# Autodesk Inventor assembly: ASY GBK короткая стенка
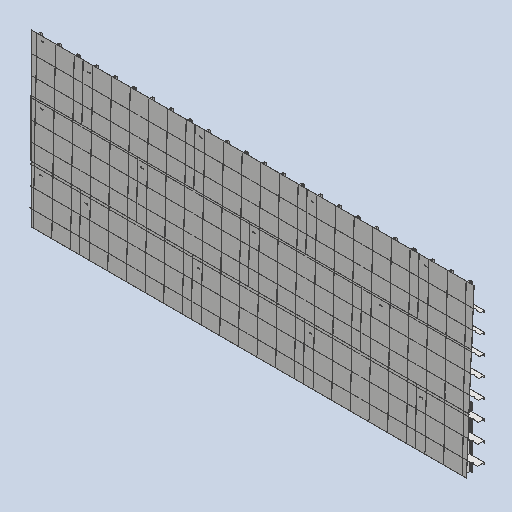
[picture p0: Inventor's stored thumbnail of the model, 512x512]
Saved by Autodesk Inventor 2026.3 (Build 303398000, 398)
## iProperties
Created: 2026-05-24
Part Number: ASY GBK короткая стенка
Document SubType Name: Assembly
Designer: pokla
Mass: 2.92121e+06 g
Surface Area: 1.88753e+06 cm^2
Volume: 372128 cm^3
Density: 7.85 g/cm^3
Stock Number: 2000
Author: pokla
## Documents named in this file (10)
- C:\Users\admin\Documents\Inventor\GBK-Gubkinskiy\ASY GBK короткая стенка.iam
- C:\Users\admin\Documents\Inventor\GBK-Gubkinskiy\ASY GBK 2110 short wall shield 1.iam
- C:\Users\admin\Documents\Inventor\GBK-Gubkinskiy\ASY GBK 2120 short wall shield 2.iam
- C:\Users\admin\Documents\Inventor\GBK-Gubkinskiy\ASY GBK 2130 short wall shield 3.iam
- C:\Users\admin\Documents\Inventor\GBK-Gubkinskiy\ASY GBK 2210 short wall shield 4.iam
- C:\Users\admin\Documents\Inventor\GBK-Gubkinskiy\ASY GBK 2310 short wall shield 7.iam
- C:\Users\admin\Documents\Inventor\GBK-Gubkinskiy\ASY GBK 2320 short wall shield 8.iam
- C:\Users\admin\Documents\Inventor\GBK-Gubkinskiy\ASY GBK 2330 short wall shield 9.iam
- C:\Users\admin\Documents\Inventor\GBK-Gubkinskiy\ASY GBK 2220 short wall shield 5.iam
- C:\Users\admin\Documents\Inventor\GBK-Gubkinskiy\ASY GBK 2230 short wall shield 6.iam
## Components (14 placed, 9 different names)
1. ASY GBK 2110 short wall shield 1:1 [sub-assembly] — Rigid:1, Flush:1, Flush:2, Mate:1
2. ASY GBK 2120 short wall shield 2:1 [sub-assembly] — Rigid:1, Rigid:2
3. ASY GBK 2120 short wall shield 2:2 [sub-assembly] — Rigid:2, Rigid:3
4. ASY GBK 2120 short wall shield 2:3 [sub-assembly] — Rigid:3, Rigid:14
5. ASY GBK 2130 short wall shield 3:1 [sub-assembly] — Rigid:14, Flush:3, Mate:2, Mate:4
6. ASY GBK 2210 short wall shield 4:1 [sub-assembly] — Rigid:17
7. ASY GBK 2220 short wall shield 5:1 [sub-assembly] — Rigid:7, Rigid:17
8. ASY GBK 2220 short wall shield 5:2 [sub-assembly] — Rigid:7, Rigid:16
9. ASY GBK 2230 short wall shield 6:1 [sub-assembly] — Flush:3, Mate:2, Flush:5, Mate:3, Mate:4, Mate:5, Rigid:16
10. ASY GBK 2310 short wall shield 7:1 [sub-assembly] — Rigid:10
11. ASY GBK 2320 short wall shield 8:1 [sub-assembly] — Rigid:10, Rigid:11
12. ASY GBK 2330 short wall shield 9:1 [sub-assembly] — Flush:5, Mate:3, Mate:5, Rigid:15
13. ASY GBK 2320 short wall shield 8:2 [sub-assembly] — Rigid:11, Rigid:12
14. ASY GBK 2320 short wall shield 8:3 [sub-assembly] — Rigid:12, Rigid:15
## Relationships (20: WeldJoint 11, Mate 5, Flush 4)
- Rigid:1 [WeldJoint] (1 mm): ASY GBK 2110 short wall shield 1:1 ↔ ASY GBK 2120 short wall shield 2:1
- Rigid:2 [WeldJoint] (1 mm): ASY GBK 2120 short wall shield 2:1 ↔ ASY GBK 2120 short wall shield 2:2
- Rigid:3 [WeldJoint] (1 mm): ASY GBK 2120 short wall shield 2:2 ↔ ASY GBK 2120 short wall shield 2:3
- Rigid:7 [WeldJoint] (1 mm): ASY GBK 2220 short wall shield 5:1 ↔ ASY GBK 2220 short wall shield 5:2
- Rigid:10 [WeldJoint] (1 mm): ASY GBK 2310 short wall shield 7:1 ↔ ASY GBK 2320 short wall shield 8:1
- Rigid:11 [WeldJoint] (1 mm): ASY GBK 2320 short wall shield 8:1 ↔ ASY GBK 2320 short wall shield 8:2
- Rigid:12 [WeldJoint] (1 mm): ASY GBK 2320 short wall shield 8:2 ↔ ASY GBK 2320 short wall shield 8:3
- Flush:1: ASY GBK 2110 short wall shield 1:1
- Flush:2: ASY GBK 2110 short wall shield 1:1
- Mate:1: ASY GBK 2110 short wall shield 1:1
- Rigid:14 [WeldJoint] (1 mm): ASY GBK 2120 short wall shield 2:3 ↔ ASY GBK 2130 short wall shield 3:1
- Flush:3: ASY GBK 2130 short wall shield 3:1 ↔ ASY GBK 2230 short wall shield 6:1
- Mate:2 (1 mm): ASY GBK 2130 short wall shield 3:1 ↔ ASY GBK 2230 short wall shield 6:1
- Flush:5: ASY GBK 2230 short wall shield 6:1 ↔ ASY GBK 2330 short wall shield 9:1
- Mate:3 (1 mm): ASY GBK 2230 short wall shield 6:1 ↔ ASY GBK 2330 short wall shield 9:1
- Mate:4 (1 mm): ASY GBK 2130 short wall shield 3:1 ↔ ASY GBK 2230 short wall shield 6:1
- Mate:5 (1 mm): ASY GBK 2230 short wall shield 6:1 ↔ ASY GBK 2330 short wall shield 9:1
- Rigid:15 [WeldJoint] (1 mm): ASY GBK 2330 short wall shield 9:1 ↔ ASY GBK 2320 short wall shield 8:3
- Rigid:16 [WeldJoint] (1 mm): ASY GBK 2220 short wall shield 5:2 ↔ ASY GBK 2230 short wall shield 6:1
- Rigid:17 [WeldJoint] (1 mm): ASY GBK 2210 short wall shield 4:1 ↔ ASY GBK 2220 short wall shield 5:1
